# Autodesk Inventor assembly: złożenie pod symulację
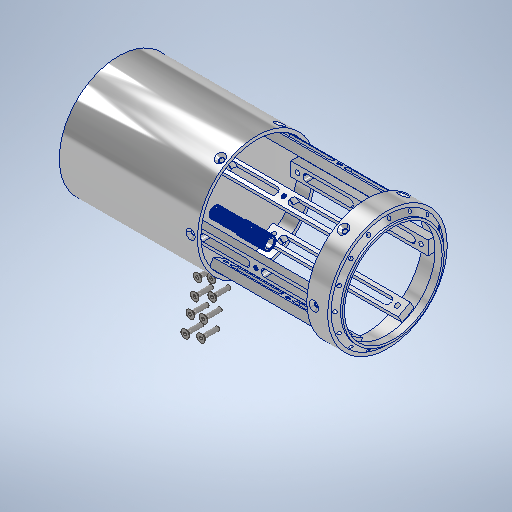
[picture p0: Inventor's stored thumbnail of the model, 512x512]
Saved by Autodesk Inventor 2025.1 (Build 291241020, 241B)
## iProperties
Created: 2024-11-05
Part Number: złożenie pod symulację
Document SubType Name: Assembly
Designer: oem
Author: oem
## Documents named in this file (5)
- C:\Users\oem\Documents\projekty\X simba\złożenie pod symulację.iam
- C:\Users\oem\Documents\projekty\X simba\R7_ENG_2000_OxidizerTank\R7_ENG_2000_OxidizerTank\R7_ENG_2000_OxidizerTank.ipt
- C:\Users\oem\Documents\projekty\X simba\R7_ENG_3101_Bracket\R7_ENG_3101_Bracket\R7_ENG_3101_Bracket.ipt
- C:\Users\oem\Documents\projekty\X simba\Radax prot 3-2\Radax prot 3-2\Radax prot 3-2.ipt
- C:\Users\oem\Documents\Inventor\Content Center Files\R2025\pl-PL\DIN 7991(2)\DIN 7991 - M6x25.ipt
## Components (20 placed, 4 different names)
1. R7_ENG_2000_OxidizerTank:1 — Zestawiające:1, Zestawiające:2
2. Radax prot 3-2:1 — Zestawiające:3, Zestawiające:4
3. DIN 7991 M6x25:1
4. DIN 7991 M6x25:2
5. DIN 7991 M6x25:3
6. DIN 7991 M6x25:4
7. DIN 7991 M6x25:5
8. DIN 7991 M6x25:6
9. DIN 7991 M6x25:7
10. DIN 7991 M6x25:8
11. DIN 7991 M6x25:9
12. DIN 7991 M6x25:10
13. DIN 7991 M6x25:11
14. DIN 7991 M6x25:12
15. R7_ENG_3101_Bracket:1 — Zestawiające:1, Zestawiające:2
16. R7_ENG_3101_Bracket:2
17. R7_ENG_3101_Bracket:3
18. R7_ENG_3101_Bracket:4 — Zestawiające:4
19. R7_ENG_3101_Bracket:5 — Zestawiające:3
20. R7_ENG_3101_Bracket:6
## Component patterns: (6 elements, first: R7_ENG_3101_Bracket:1)
## Relationships (4: Mate 4)
- Zestawiające:1 [Mate]: R7_ENG_2000_OxidizerTank:1 ↔ R7_ENG_3101_Bracket:1
- Zestawiające:2 [Mate]: R7_ENG_2000_OxidizerTank:1 ↔ R7_ENG_3101_Bracket:1
- Zestawiające:3 [Mate]: Radax prot 3-2:1 ↔ R7_ENG_3101_Bracket:5
- Zestawiające:4 [Mate]: Radax prot 3-2:1 ↔ R7_ENG_3101_Bracket:4
